# Autodesk Inventor assembly: motor+gbox assembly
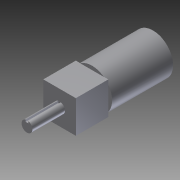
[picture p0: Inventor's stored thumbnail of the model, 180x180]
Saved by Autodesk Inventor 2011 SP1 (Build 150282100, 282)
## iProperties
Created: 2013-01-16
Part Number: motor+gbox assembly
Document SubType Name: Assembly
Designer: 961407
Author: 961407
## Documents named in this file (3)
- \\WW427-DATA1\StuHome\961407\Documents\GitHub\2013CAD\2013 robot\CurvedShooter\motor+gbox assembly.iam
- \\WW427-DATA1\StuHome\961407\Documents\GitHub\2013CAD\2013 robot\CurvedShooter\RS775 18v.ipt
- \\WW427-DATA1\StuHome\961407\Documents\GitHub\2013CAD\2013 robot\CurvedShooter\BaneBots P60 4 to1 gearbox.ipt
## Components (2 placed, 2 different names)
1. RS775 18v:1 — Insert:1
2. BaneBots P60 4 to1 gearbox:1 — Insert:1
## Relationships (1: Insert 1)
- Insert:1: RS775 18v:1 ↔ BaneBots P60 4 to1 gearbox:1
